# Autodesk Inventor assembly: 000-belt_liner_v3
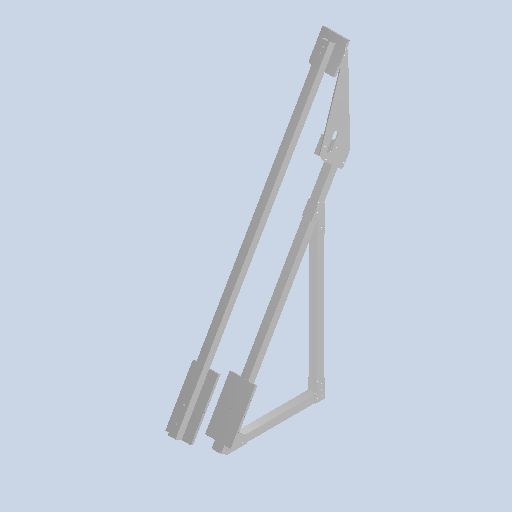
[picture p0: Inventor's stored thumbnail of the model, 512x512]
Saved by Autodesk Inventor 2025.2 (Build 292293000, 293)
## iProperties
Created: 2025-01-19
Part Number: 000-belt_liner_v3
Document SubType Name: Assembly
Designer: haruy
Author: haruy
## Documents named in this file (10)
- C:\Users\haruy\Documents\ロボコン\NHK2025\cad\nagahisa\belt_liner\000-belt_liner_v3.iam
- C:\Users\haruy\Documents\ロボコン\NHK2025\cad\nagahisa\belt_liner\belt_liner_v3_ASP_Base.ipt
- C:\Users\haruy\Documents\ロボコン\NHK2025\cad\nagahisa\belt_liner\belt_liner_v1_Plate_12.ipt
- C:\Users\haruy\Documents\ロボコン\NHK2025\cad\nagahisa\belt_liner\belt_liner_v3_Plate_1.ipt
- C:\Users\haruy\Documents\ロボコン\NHK2025\cad\nagahisa\belt_liner\belt_liner_v3_Plate_2.ipt
- C:\Users\haruy\Documents\ロボコン\NHK2025\cad\nagahisa\belt_liner\belt_liner_v2_Plate_10.ipt
- C:\Users\haruy\Documents\ロボコン\NHK2025\cad\nagahisa\belt_liner\belt_liner_v2_Plate_11.ipt
- C:\Users\haruy\Documents\ロボコン\NHK2025\cad\nagahisa\belt_liner\belt_liner_v2_Plate_2.ipt
- C:\Users\haruy\Documents\ロボコン\NHK2025\cad\nagahisa\belt_liner\belt_liner_v2_Plate_9.ipt
- C:\Users\haruy\Documents\ロボコン\NHK2025\cad\nagahisa\belt_liner\belt_liner_v2_Plate_8.ipt
## Components (12 placed, 9 different names)
1. belt_liner_v3_ASP_Base:1 — 挿入:1, 挿入:2, 挿入:3, 挿入:4, 挿入:5, 挿入:6, 挿入:7, 挿入:8, 挿入:9, 挿入:10, 挿入:11, 挿入:12, 挿入:13, 挿入:14, 挿入:15, 挿入:16, 挿入:19, 挿入:20, 挿入:21, 挿入:22
2. belt_liner_v1_Plate_12:1 — 挿入:1, 挿入:2
3. belt_liner_v1_Plate_12:2 — 挿入:3, 挿入:4
4. belt_liner_v3_Plate_1:1 — 挿入:5, 挿入:6
5. belt_liner_v3_Plate_1:2 — 挿入:7, 挿入:8
6. belt_liner_v3_Plate_2:1 — 挿入:9, 挿入:10
7. belt_liner_v3_Plate_2:2 — 挿入:11, 挿入:12
8. belt_liner_v2_Plate_10:1 — 挿入:13, 挿入:14, 挿入:18
9. belt_liner_v2_Plate_11:1 — 挿入:15, 挿入:16, 挿入:17
10. belt_liner_v2_Plate_2:1 — 挿入:17, 挿入:18
11. belt_liner_v2_Plate_9:1 — 挿入:19, 挿入:20
12. belt_liner_v2_Plate_8:1 — 挿入:21, 挿入:22
## Relationships (22: Insert 22)
- 挿入:1 [Insert]: belt_liner_v3_ASP_Base:1 ↔ belt_liner_v1_Plate_12:1
- 挿入:2 [Insert]: belt_liner_v3_ASP_Base:1 ↔ belt_liner_v1_Plate_12:1
- 挿入:3 [Insert]: belt_liner_v3_ASP_Base:1 ↔ belt_liner_v1_Plate_12:2
- 挿入:4 [Insert]: belt_liner_v3_ASP_Base:1 ↔ belt_liner_v1_Plate_12:2
- 挿入:5 [Insert]: belt_liner_v3_ASP_Base:1 ↔ belt_liner_v3_Plate_1:1
- 挿入:6 [Insert]: belt_liner_v3_ASP_Base:1 ↔ belt_liner_v3_Plate_1:1
- 挿入:7 [Insert]: belt_liner_v3_ASP_Base:1 ↔ belt_liner_v3_Plate_1:2
- 挿入:8 [Insert]: belt_liner_v3_ASP_Base:1 ↔ belt_liner_v3_Plate_1:2
- 挿入:9 [Insert]: belt_liner_v3_ASP_Base:1 ↔ belt_liner_v3_Plate_2:1
- 挿入:10 [Insert]: belt_liner_v3_ASP_Base:1 ↔ belt_liner_v3_Plate_2:1
- 挿入:11 [Insert]: belt_liner_v3_ASP_Base:1 ↔ belt_liner_v3_Plate_2:2
- 挿入:12 [Insert]: belt_liner_v3_ASP_Base:1 ↔ belt_liner_v3_Plate_2:2
- 挿入:13 [Insert]: belt_liner_v3_ASP_Base:1 ↔ belt_liner_v2_Plate_10:1
- 挿入:14 [Insert]: belt_liner_v3_ASP_Base:1 ↔ belt_liner_v2_Plate_10:1
- 挿入:15 [Insert]: belt_liner_v3_ASP_Base:1 ↔ belt_liner_v2_Plate_11:1
- 挿入:16 [Insert]: belt_liner_v3_ASP_Base:1 ↔ belt_liner_v2_Plate_11:1
- 挿入:17 [Insert]: belt_liner_v2_Plate_11:1 ↔ belt_liner_v2_Plate_2:1
- 挿入:18 [Insert]: belt_liner_v2_Plate_10:1 ↔ belt_liner_v2_Plate_2:1
- 挿入:19 [Insert]: belt_liner_v3_ASP_Base:1 ↔ belt_liner_v2_Plate_9:1
- 挿入:20 [Insert]: belt_liner_v3_ASP_Base:1 ↔ belt_liner_v2_Plate_9:1
- 挿入:21 [Insert]: belt_liner_v3_ASP_Base:1 ↔ belt_liner_v2_Plate_8:1
- 挿入:22 [Insert]: belt_liner_v3_ASP_Base:1 ↔ belt_liner_v2_Plate_8:1
